# Autodesk Inventor assembly: kicker
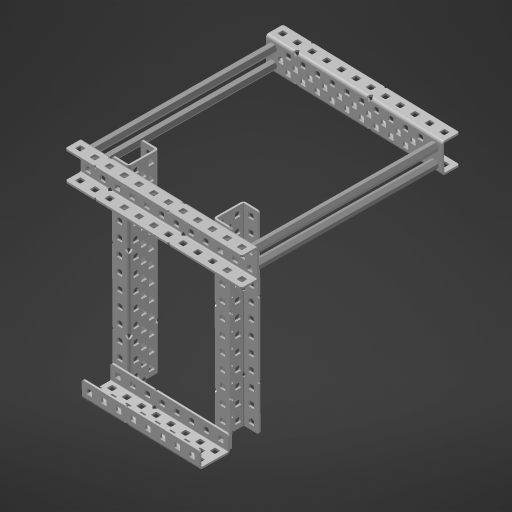
[picture p0: Inventor's stored thumbnail of the model, 512x512]
Saved by Autodesk Inventor 2024 (Build 280153000, 153)
## iProperties
Created: 2023-11-26
Part Number: kicker
Document SubType Name: Assembly
Designer: Meer
Author: Meer
## Documents named in this file (7)
- C:\Users\Meer\OneDrive\Documents\GitHub\2023-599Z\BBotCAD\kicker.iam
- C:\Users\Meer\OneDrive\Documents\GitHub\2023-599Z\BBotCAD\VEX-CAD-Inventor-1.4.0\Structure\C Channel\Aluminum 1x2x1\Alu C 1x2x1x20.ipt
- C:\Users\Meer\OneDrive\Documents\GitHub\2023-599Z\BBotCAD\VEX-CAD-Inventor-1.4.0\Structure\Standoff.ipt
- C:\Users\Meer\OneDrive\Documents\GitHub\2023-599Z\BBotCAD\VEX-CAD-Inventor-1.4.0\Structure\Standoff\Standoff 6.00.ipt
- C:\Users\Meer\OneDrive\Documents\GitHub\2023-599Z\BBotCAD\VEX-CAD-Inventor-1.4.0\Structure\C Channel\Aluminum 1x2x1\Alu C 1x2x1x12.ipt
- C:\Users\Meer\OneDrive\Documents\GitHub\2023-599Z\BBotCAD\VEX-CAD-Inventor-1.4.0\Structure\C Channel\Aluminum 1x2x1\Alu C 1x2x1x13.ipt
- C:\Users\Meer\OneDrive\Documents\GitHub\2023-599Z\BBotCAD\VEX-CAD-Inventor-1.4.0\Structure\C Channel\Aluminum 1x2x1\Alu C 1x2x1x8.ipt
## Components (10 placed, 5 different names)
1. Alu C 1x2x1x20:1
2. Standoff 6.00:1 — Insert:1, Insert:6
3. Standoff 6.00:2 — Insert:2, Insert:5
4. Standoff 6.00:3 — Insert:3
5. Standoff 6.00:4 — Insert:4
6. Alu C 1x2x1x12:3 — Insert:5, Insert:6
7. Alu C 1x2x1x12:4 — Insert:1, Insert:2, Insert:3, Insert:4, Insert:7, Insert:8, Mate:1, Insert:9
8. Alu C 1x2x1x13:1 — Insert:7, Insert:8, Insert:11
9. Alu C 1x2x1x13:2 — Mate:1, Insert:9, Insert:10
10. Alu C 1x2x1x8:1 — Insert:10, Insert:11
## Relationships (12: Insert 11, Mate 1)
- Insert:1: Standoff 6.00:1 ↔ Alu C 1x2x1x12:4
- Insert:2: Standoff 6.00:2 ↔ Alu C 1x2x1x12:4
- Insert:3: Standoff 6.00:3 ↔ Alu C 1x2x1x12:4
- Insert:4: Standoff 6.00:4 ↔ Alu C 1x2x1x12:4
- Insert:5: Standoff 6.00:2 ↔ Alu C 1x2x1x12:3
- Insert:6: Standoff 6.00:1 ↔ Alu C 1x2x1x12:3
- Insert:7: Alu C 1x2x1x12:4 ↔ Alu C 1x2x1x13:1
- Insert:8: Alu C 1x2x1x12:4 ↔ Alu C 1x2x1x13:1
- Mate:1: Alu C 1x2x1x12:4 ↔ Alu C 1x2x1x13:2
- Insert:9: Alu C 1x2x1x12:4 ↔ Alu C 1x2x1x13:2
- Insert:10: Alu C 1x2x1x13:2 ↔ Alu C 1x2x1x8:1
- Insert:11: Alu C 1x2x1x13:1 ↔ Alu C 1x2x1x8:1
